# Autodesk Inventor assembly: Printer-v2
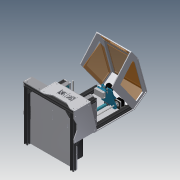
[picture p0: Inventor's stored thumbnail of the model, 180x180]
Saved by Autodesk Inventor 2014 (Build 180170000, 170)
## iProperties
Created: 2015-02-16
Part Number: Printer-v2
Document SubType Name: Assembly
Designer: Peele
Author: Peele
## Documents named in this file (18)
- E:\Copy\DLP\DMP-SL-v2\Printer-v2.iam
- E:\Copy\DLP\DMP-SL-v2\SubAssem\NewFrame.iam
- E:\Copy\DLP\DMP-SL-v2\CustomParts\ProjectorPlateFront.ipt
- E:\Copy\DLP\DMP-SL-v2\CustomParts\ProjectorPlateBack.ipt
- E:\Copy\DLP\DMP-SL-v2\CustomParts\MirrorPlate.ipt
- E:\Copy\DLP\DMP-SL-v2\CustomParts\XaxisAssem.iam
- E:\Copy\DLP\DMP-SL-v2\CustomParts\YaxisAssem.iam
- E:\Copy\DLP\DMP-SL-v2\SubAssem\PlatformAssenm.iam
- E:\Copy\DLP\DMP-SL-v2\SubAssem\NewVatAssem.iam
- E:\Copy\DLP\DMP-SL-v2\CustomParts\FrontPanel.ipt
- E:\Copy\DLP\DMP-SL-v2\CustomParts\BottomRightSide.ipt
- E:\Copy\DLP\DMP-SL-v2\CustomParts\ControlRightPanel.ipt
- E:\Copy\DLP\DMP-SL-v2\CustomParts\FrontLeft.ipt
- E:\Copy\DLP\DMP-SL-v2\CustomParts\LeftSidePanel.ipt
- E:\Copy\DLP\DMP-SL-v2\CustomParts\NewControlPanel.ipt
- E:\Copy\DLP\DMP-SL-v2\SubAssem\FrontCover.iam
- E:\Copy\DLP\DMP-SL-v2\StockParts\Projector-AcerP1500.ipt
- E:\Copy\DLP\DMP-SL-v2\StockParts\Button.ipt
## Components (19 placed, 17 different names)
1. NewFrame:1 [sub-assembly] — Flush:1, Flush:2, Flush:3, Mate:1, Flush:4, Flush:5, Mate:2, Flush:6, Flush:7, Mate:5, Flush:8, Flush:9, Mate:6, Flush:10, Flush:11, Mate:11, Flush:12, Flush:13, Flush:14, Flush:15, Mate:14, Flush:18, Mate:16, Flush:19
2. ProjectorPlateFront:1 — Mate:1, Flush:4, Flush:5, Mate:3, Mate:4, Tangent:6
3. ProjectorPlateBack:1 — Mate:2, Flush:6, Mate:3, Mate:22
4. MirrorPlate:1 — Mate:4, Flush:7, Tangent:6
5. XaxisAssem:1 [sub-assembly] — Mate:5, Flush:8, Flush:9, Mate:9, Mate:10, Mate:12, Mate:13
6. YaxisAssem:1 [sub-assembly] — Mate:6, Flush:10, Flush:11, Mate:7, Mate:8, Flush:20, Mate:21
7. PlatformAssenm:1 [sub-assembly] — Mate:7, Mate:8
8. NewVatAssem:1 [sub-assembly] — Mate:9, Mate:10
9. FrontPanel:1 — Mate:11, Flush:12, Flush:13, Flush:16, Mate:15
10. BottomRightSide:1 — Mate:12, Flush:14, Flush:15, Flush:17
11. ControlRightPanel:1 — Mate:13, Flush:16, Flush:17, Mate:19
12. FrontLeft:1 — Mate:14, Flush:18, Mate:15, Mate:17, Mate:20
13. LeftSidePanel:1 — Mate:16, Flush:19, Mate:17, Mate:18
14. NewControlPanel:1 — Mate:18, Mate:19, Mate:20, Mate:23, Mate:24, Mate:25, Mate:26
15. FrontCover:1 [sub-assembly] — Flush:20, Mate:21
16. Projector-AcerP1500:1 — Mate:22
17. Button:1 — Mate:23, Mate:26, Flush:21
18. Button:2 — Mate:24, Flush:21, Flush:22
19. Button:3 — Mate:25, Flush:22
## Relationships (49: Mate 26, Flush 22, Tangent 1)
- Flush:1: NewFrame:1
- Flush:2: NewFrame:1
- Flush:3: NewFrame:1
- Mate:1: NewFrame:1 ↔ ProjectorPlateFront:1
- Flush:4: NewFrame:1 ↔ ProjectorPlateFront:1
- Flush:5: NewFrame:1 ↔ ProjectorPlateFront:1
- Mate:2: NewFrame:1 ↔ ProjectorPlateBack:1
- Flush:6: NewFrame:1 ↔ ProjectorPlateBack:1
- Mate:3: ProjectorPlateFront:1 ↔ ProjectorPlateBack:1
- Mate:4: ProjectorPlateFront:1 ↔ MirrorPlate:1
- Flush:7 (85 mm): NewFrame:1 ↔ MirrorPlate:1
- Tangent:6: ProjectorPlateFront:1 ↔ MirrorPlate:1
- Mate:5: NewFrame:1 ↔ XaxisAssem:1
- Flush:8: NewFrame:1 ↔ XaxisAssem:1
- Flush:9: NewFrame:1 ↔ XaxisAssem:1
- Mate:6: NewFrame:1 ↔ YaxisAssem:1
- Flush:10: NewFrame:1 ↔ YaxisAssem:1
- Flush:11 (6 mm): NewFrame:1 ↔ YaxisAssem:1
- Mate:7: YaxisAssem:1 ↔ PlatformAssenm:1
- Mate:8: YaxisAssem:1 ↔ PlatformAssenm:1
- Mate:9: XaxisAssem:1 ↔ NewVatAssem:1
- Mate:10: XaxisAssem:1 ↔ NewVatAssem:1
- Mate:11: NewFrame:1 ↔ FrontPanel:1
- Flush:12: NewFrame:1 ↔ FrontPanel:1
- Flush:13 (9 mm): NewFrame:1 ↔ FrontPanel:1
- Mate:12: XaxisAssem:1 ↔ BottomRightSide:1
- Flush:14: NewFrame:1 ↔ BottomRightSide:1
- Flush:15: NewFrame:1 ↔ BottomRightSide:1
- Mate:13: XaxisAssem:1 ↔ ControlRightPanel:1
- Flush:16: FrontPanel:1 ↔ ControlRightPanel:1
- Flush:17: BottomRightSide:1 ↔ ControlRightPanel:1
- Mate:14: NewFrame:1 ↔ FrontLeft:1
- Flush:18: NewFrame:1 ↔ FrontLeft:1
- Mate:15: FrontPanel:1 ↔ FrontLeft:1
- Mate:16: NewFrame:1 ↔ LeftSidePanel:1
- Flush:19: NewFrame:1 ↔ LeftSidePanel:1
- Mate:17: FrontLeft:1 ↔ LeftSidePanel:1
- Mate:18: LeftSidePanel:1 ↔ NewControlPanel:1
- Mate:19: ControlRightPanel:1 ↔ NewControlPanel:1
- Mate:20: FrontLeft:1 ↔ NewControlPanel:1
- Flush:20: YaxisAssem:1 ↔ FrontCover:1
- Mate:21: YaxisAssem:1 ↔ FrontCover:1
- Mate:22: ProjectorPlateBack:1 ↔ Projector-AcerP1500:1
- Mate:23: NewControlPanel:1 ↔ Button:1
- Mate:24: NewControlPanel:1 ↔ Button:2
- Mate:25: NewControlPanel:1 ↔ Button:3
- Mate:26: NewControlPanel:1 ↔ Button:1
- Flush:21: Button:1 ↔ Button:2
- Flush:22: Button:2 ↔ Button:3
